# Autodesk Inventor assembly: PnumaticActiveClimb-ver3-1111-2021
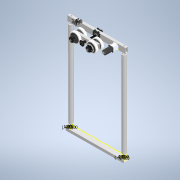
[picture p0: Inventor's stored thumbnail of the model, 180x180]
Saved by Autodesk Inventor 2021 (Build 250183000, 183)
## iProperties
Created: 2021-01-28
Part Number: PnumaticActiveClimb-ver3-1111-2021
Document SubType Name: Assembly
Designer: CMurray
Author: CMurray
## Documents named in this file (19)
- E:\PHRC CADD 2021\PHRC CADD\2020 Infinite Recharge\2021 Infinite Recharge\Chassis\PnumaticActiveClimb-ver3-1111-2021.iam
- E:\PHRC CADD 2021\PHRC CADD\2020 Infinite Recharge\Active Climb\Parts\2x1 16in Aluminum-ver1-1111-2020.ipt
- E:\PHRC CADD 2021\PHRC CADD\Resources\VEXpro Resources\Versa Motion\VersaBlockKit-1111-2016.ipt
- E:\PHRC CADD 2021\PHRC CADD\Resources\VEXpro Resources\Bearings\0.5inHexFlangedBearing(1.125inx0.313in)-1111-2016.ipt
- E:\PHRC CADD 2021\PHRC CADD\Resources\VEXpro Resources\Shafts\0.5inThunderHexShaft(8in(modified))-1111-2016.ipt
- E:\PHRC CADD 2021\PHRC CADD\2020 Infinite Recharge\Active Climb\Parts\AluminumBar-1111-2020.ipt
- E:\PHRC CADD 2021\PHRC CADD\Resources\VEXpro Resources\Spacers\1inAcetalSpacer(0.5inHex)-1111-2016.ipt
- E:\PHRC CADD 2021\PHRC CADD\Resources\VEXpro Resources\Versa Motion\Sprockets\Sprocket15t-ver1-1111-2017.ipt
- E:\PHRC CADD 2021\PHRC CADD\Resources\VEXpro Resources\Versa Motion\Shaft Collars\ClampingShaftCollar0.5inHex-ver1-1111-2017.ipt
- E:\PHRC CADD 2021\PHRC CADD\Resources\VEXpro Resources\Shafts\0.5inThunderHexShaft(8)-1111-2016.ipt
- E:\PHRC CADD 2021\PHRC CADD\Resources\VEXpro Resources\Wheels\4 inch\4inColsonPerformaWheel-1111-2017.ipt
- E:\PHRC CADD 2021\PHRC CADD\Resources\VEXpro Resources\Spacers\.25inchromatesteelwasher-1111-2018.ipt
- E:\PHRC CADD 2021\PHRC CADD\Resources\VEXpro Resources\Versa Motion\Sprockets\1.125HexboreSprocket22t-ver-1111-2018.ipt
- E:\PHRC CADD 2021\PHRC CADD\Resources\VEXpro Resources\Versa Motion\VersaHub(0.5inHex)-1111-2016.ipt
- E:\PHRC CADD 2021\PHRC CADD\Resources\VEXpro Resources\Spacers\0.0625inAcetalSpacer(0.5inHex)-1111-2016.ipt
- E:\PHRC CADD 2021\PHRC CADD\Resources\VEXpro Resources\Spacers\1inAcetalSpacer(0.5inHex)-1111-2016_MIR.ipt
- E:\PHRC CADD 2021\PHRC CADD\Resources\VEXpro Resources\Motors\v2-VersaPlanetary-3in-1stage-with-775pro-20161031.iam
- E:\PHRC CADD 2021\PHRC CADD\2020 Infinite Recharge\Lift\Parts\1.5_Bore_30in_Stroke_ROUND BODY AIR CYLINDER.iam
- E:\PHRC CADD 2021\PHRC CADD\2020 Infinite Recharge\Lift\Assemblies\ClimbBase-1111-2020.iam
## Components (39 placed, 18 different names)
1. 2x1 16in Aluminum-ver1-1111-2020:1 — Rotational:1, Angle:1, Rotational:2, Angle:2, Mate:1, Flush:1, Flush:2, Cylindrical:21, Mate:24, Angle:26, Flush:7, Flush:8, Mate:25
2. VersaBlockKit-1111-2016:1 — Rotational:1, Angle:1, Rotational:3
3. VersaBlockKit-1111-2016:2 — Rotational:2, Angle:2, Rotational:4
4. 0.5inHexFlangedBearing(1.125inx0.313in)-1111-2016:1 — Rotational:3, Cylindrical:1, Angle:6
5. 0.5inHexFlangedBearing(1.125inx0.313in)-1111-2016:2 — Rotational:4, Angle:7
6. 0.5inThunderHexShaft(8in(modified))-1111-2016:1 — Cylindrical:1, Angle:5, Angle:6, Angle:7, Cylindrical:3, Angle:8, Cylindrical:4, Flush:3, Angle:24, Angle:25
7. AluminumBar-1111-2020:1 — Mate:1, Flush:1, Flush:2, Rotational:5, Rotational:6, Flush:3, Rotational:7, Rotational:8, Rotational:9, Rotational:10, Flush:4, Mate:7, Flush:5
8. 0.5inHexFlangedBearing(1.125inx0.313in)-1111-2016:3 — Rotational:5, Cylindrical:2, Mate:2, Angle:3, Angle:4
9. 0.5inHexFlangedBearing(1.125inx0.313in)-1111-2016:4 — Rotational:6, Angle:3, Angle:5
10. 1inAcetalSpacer(0.5inHex)-1111-2016:1 — Cylindrical:2, Mate:2, Angle:4, Mate:3
11. Sprocket15t-ver1-1111-2017:1 — Cylindrical:3, Mate:3, Angle:8, Mate:4
12. ClampingShaftCollar0.5inHex-ver1-1111-2017:1 — Cylindrical:4, Mate:4
13. 0.5inHexFlangedBearing(1.125inx0.313in)-1111-2016:5 — Rotational:7, Cylindrical:5, Angle:9, Mate:17
14. 0.5inHexFlangedBearing(1.125inx0.313in)-1111-2016:6 — Rotational:8, Angle:10, Mate:5
15. 0.5inHexFlangedBearing(1.125inx0.313in)-1111-2016:7 — Rotational:9, Cylindrical:14, Angle:18, Mate:20
16. 0.5inHexFlangedBearing(1.125inx0.313in)-1111-2016:8 — Rotational:10, Angle:19, Mate:18
17. 0.5inThunderHexShaft(8)-1111-2016:1 — Cylindrical:5, Angle:9, Angle:10, Cylindrical:6, Angle:11, Cylindrical:7, Flush:4, Cylindrical:8, Angle:12, Cylindrical:9, Angle:15, Cylindrical:10, Angle:16, Cylindrical:11, Cylindrical:12, Cylindrical:13, Angle:17, Angle:25
18. 4inColsonPerformaWheel-1111-2017:1 — Cylindrical:6, Mate:5, Angle:11, Mate:6
19. .25inchromatesteelwasher-1111-2018:1 — Cylindrical:7, Mate:6
20. 1.125HexboreSprocket22t-ver-1111-2018:1 — Rotational:11, Mate:7, Mate:16
21. VersaHub(0.5inHex)-1111-2016:2 — Rotational:11, Cylindrical:8, Angle:12, Mate:12, Mate:16
22. 0.0625inAcetalSpacer(0.5inHex)-1111-2016:1 — Mate:8, Mate:9, Cylindrical:9, Angle:13, Angle:15, Mate:12
23. 0.0625inAcetalSpacer(0.5inHex)-1111-2016:2 — Mate:8, Mate:9, Mate:10, Mate:11, Angle:13, Angle:14
24. 0.0625inAcetalSpacer(0.5inHex)-1111-2016:3 — Mate:10, Mate:11, Angle:14, Mate:13
25. Sprocket15t-ver1-1111-2017:2 — Cylindrical:10, Angle:16, Mate:13, Mate:14
26. ClampingShaftCollar0.5inHex-ver1-1111-2017:2 — Cylindrical:11, Mate:14, Mate:15
27. .25inchromatesteelwasher-1111-2018:2 — Cylindrical:12, Mate:15
28. 4inColsonPerformaWheel-1111-2017:2 — Cylindrical:13, Mate:17, Angle:17
29. 0.5inThunderHexShaft(8)-1111-2016:2 — Cylindrical:14, Angle:18, Angle:19, Flush:5, Cylindrical:15, Angle:20, Cylindrical:16, Cylindrical:17, Angle:21, Cylindrical:18, Angle:22, Cylindrical:19, Angle:23, Cylindrical:20, Angle:24
30. 4inColsonPerformaWheel-1111-2017:3 — Cylindrical:15, Mate:18, Angle:20, Mate:19
31. .25inchromatesteelwasher-1111-2018:3 — Cylindrical:16, Mate:19
32. 4inColsonPerformaWheel-1111-2017:4 — Cylindrical:17, Mate:20, Angle:21, Mate:21
33. 1inAcetalSpacer(0.5inHex)-1111-2016_MIR:1 — Cylindrical:18, Mate:21, Angle:22, Mate:22
34. Sprocket15t-ver1-1111-2017:3 — Cylindrical:19, Mate:22, Angle:23, Mate:23
35. .25inchromatesteelwasher-1111-2018:4 — Cylindrical:20, Mate:23
36. v2-VersaPlanetary-3in-1stage-with-775pro-20161031:1 [sub-assembly] — Cylindrical:21, Mate:24, Angle:26
37. 1.5_Bore_30in_Stroke_ROUND BODY AIR CYLINDER:3 [sub-assembly] — Flush:6
38. 1.5_Bore_30in_Stroke_ROUND BODY AIR CYLINDER:4 [sub-assembly] — Rotational:12, Flush:6
39. ClimbBase-1111-2020:2 [sub-assembly] — Rotational:12, Flush:7, Flush:8, Mate:25
## Relationships (93: Angle 26, Mate 25, CylindricalJoint 21, RevoluteJoint 12, Flush 8, Insert 1)
- Rotational:1 [RevoluteJoint]: 2x1 16in Aluminum-ver1-1111-2020:1 ↔ VersaBlockKit-1111-2016:1
- Angle:1 (0 deg): 2x1 16in Aluminum-ver1-1111-2020:1 ↔ VersaBlockKit-1111-2016:1
- Rotational:2 [RevoluteJoint]: 2x1 16in Aluminum-ver1-1111-2020:1 ↔ VersaBlockKit-1111-2016:2
- Angle:2 (0 deg): 2x1 16in Aluminum-ver1-1111-2020:1 ↔ VersaBlockKit-1111-2016:2
- Rotational:3 [RevoluteJoint]: VersaBlockKit-1111-2016:1 ↔ 0.5inHexFlangedBearing(1.125inx0.313in)-1111-2016:1
- Rotational:4 [RevoluteJoint]: VersaBlockKit-1111-2016:2 ↔ 0.5inHexFlangedBearing(1.125inx0.313in)-1111-2016:2
- Cylindrical:1: 0.5inHexFlangedBearing(1.125inx0.313in)-1111-2016:1 ↔ 0.5inThunderHexShaft(8in(modified))-1111-2016:1
- Mate:1 (85.725 mm): 2x1 16in Aluminum-ver1-1111-2020:1 ↔ AluminumBar-1111-2020:1
- Flush:1: 2x1 16in Aluminum-ver1-1111-2020:1 ↔ AluminumBar-1111-2020:1
- Flush:2 (174.625 mm): 2x1 16in Aluminum-ver1-1111-2020:1 ↔ AluminumBar-1111-2020:1
- Rotational:5 [RevoluteJoint]: AluminumBar-1111-2020:1 ↔ 0.5inHexFlangedBearing(1.125inx0.313in)-1111-2016:3
- Rotational:6 [RevoluteJoint]: AluminumBar-1111-2020:1 ↔ 0.5inHexFlangedBearing(1.125inx0.313in)-1111-2016:4
- Cylindrical:2: 0.5inHexFlangedBearing(1.125inx0.313in)-1111-2016:3 ↔ 1inAcetalSpacer(0.5inHex)-1111-2016:1
- Mate:2: 0.5inHexFlangedBearing(1.125inx0.313in)-1111-2016:3 ↔ 1inAcetalSpacer(0.5inHex)-1111-2016:1
- Angle:3 (0 deg): 0.5inHexFlangedBearing(1.125inx0.313in)-1111-2016:3 ↔ 0.5inHexFlangedBearing(1.125inx0.313in)-1111-2016:4
- Angle:4 (0 deg): 0.5inHexFlangedBearing(1.125inx0.313in)-1111-2016:3 ↔ 1inAcetalSpacer(0.5inHex)-1111-2016:1
- Angle:5 (90 deg): 0.5inThunderHexShaft(8in(modified))-1111-2016:1 ↔ 0.5inHexFlangedBearing(1.125inx0.313in)-1111-2016:4
- Angle:6 (90 deg): 0.5inHexFlangedBearing(1.125inx0.313in)-1111-2016:1 ↔ 0.5inThunderHexShaft(8in(modified))-1111-2016:1
- Angle:7 (90 deg): 0.5inHexFlangedBearing(1.125inx0.313in)-1111-2016:2 ↔ 0.5inThunderHexShaft(8in(modified))-1111-2016:1
- Cylindrical:3: 0.5inThunderHexShaft(8in(modified))-1111-2016:1 ↔ Sprocket15t-ver1-1111-2017:1
- Mate:3: 1inAcetalSpacer(0.5inHex)-1111-2016:1 ↔ Sprocket15t-ver1-1111-2017:1
- Angle:8 (90 deg): 0.5inThunderHexShaft(8in(modified))-1111-2016:1 ↔ Sprocket15t-ver1-1111-2017:1
- Cylindrical:4: 0.5inThunderHexShaft(8in(modified))-1111-2016:1 ↔ ClampingShaftCollar0.5inHex-ver1-1111-2017:1
- Mate:4: Sprocket15t-ver1-1111-2017:1 ↔ ClampingShaftCollar0.5inHex-ver1-1111-2017:1
- Flush:3 (50.8 mm): 0.5inThunderHexShaft(8in(modified))-1111-2016:1 ↔ AluminumBar-1111-2020:1
- Rotational:7 [RevoluteJoint]: AluminumBar-1111-2020:1 ↔ 0.5inHexFlangedBearing(1.125inx0.313in)-1111-2016:5
- Rotational:8 [RevoluteJoint]: AluminumBar-1111-2020:1 ↔ 0.5inHexFlangedBearing(1.125inx0.313in)-1111-2016:6
- Rotational:9 [RevoluteJoint]: AluminumBar-1111-2020:1 ↔ 0.5inHexFlangedBearing(1.125inx0.313in)-1111-2016:7
- Rotational:10 [RevoluteJoint]: AluminumBar-1111-2020:1 ↔ 0.5inHexFlangedBearing(1.125inx0.313in)-1111-2016:8
- Cylindrical:5: 0.5inHexFlangedBearing(1.125inx0.313in)-1111-2016:5 ↔ 0.5inThunderHexShaft(8)-1111-2016:1
- Angle:9 (90 deg): 0.5inHexFlangedBearing(1.125inx0.313in)-1111-2016:5 ↔ 0.5inThunderHexShaft(8)-1111-2016:1
- Angle:10 (90 deg): 0.5inHexFlangedBearing(1.125inx0.313in)-1111-2016:6 ↔ 0.5inThunderHexShaft(8)-1111-2016:1
- Cylindrical:6: 0.5inThunderHexShaft(8)-1111-2016:1 ↔ 4inColsonPerformaWheel-1111-2017:1
- Mate:5: 0.5inHexFlangedBearing(1.125inx0.313in)-1111-2016:6 ↔ 4inColsonPerformaWheel-1111-2017:1
- Angle:11 (90 deg): 0.5inThunderHexShaft(8)-1111-2016:1 ↔ 4inColsonPerformaWheel-1111-2017:1
- Cylindrical:7: 0.5inThunderHexShaft(8)-1111-2016:1 ↔ .25inchromatesteelwasher-1111-2018:1
- Mate:6: 4inColsonPerformaWheel-1111-2017:1 ↔ .25inchromatesteelwasher-1111-2018:1
- Flush:4 (38.1 mm): AluminumBar-1111-2020:1 ↔ 0.5inThunderHexShaft(8)-1111-2016:1
- Rotational:11 [RevoluteJoint]: 1.125HexboreSprocket22t-ver-1111-2018:1 ↔ VersaHub(0.5inHex)-1111-2016:2
- Cylindrical:8: 0.5inThunderHexShaft(8)-1111-2016:1 ↔ VersaHub(0.5inHex)-1111-2016:2
- Mate:7 (34.925 mm): AluminumBar-1111-2020:1 ↔ 1.125HexboreSprocket22t-ver-1111-2018:1
- Mate:8: 0.0625inAcetalSpacer(0.5inHex)-1111-2016:1 ↔ 0.0625inAcetalSpacer(0.5inHex)-1111-2016:2
- Mate:9: 0.0625inAcetalSpacer(0.5inHex)-1111-2016:1 ↔ 0.0625inAcetalSpacer(0.5inHex)-1111-2016:2
- Mate:10: 0.0625inAcetalSpacer(0.5inHex)-1111-2016:2 ↔ 0.0625inAcetalSpacer(0.5inHex)-1111-2016:3
- Mate:11: 0.0625inAcetalSpacer(0.5inHex)-1111-2016:2 ↔ 0.0625inAcetalSpacer(0.5inHex)-1111-2016:3
- Angle:12 (90 deg): 0.5inThunderHexShaft(8)-1111-2016:1 ↔ VersaHub(0.5inHex)-1111-2016:2
- Cylindrical:9: 0.5inThunderHexShaft(8)-1111-2016:1 ↔ 0.0625inAcetalSpacer(0.5inHex)-1111-2016:1
- Angle:13 (0 deg): 0.0625inAcetalSpacer(0.5inHex)-1111-2016:1 ↔ 0.0625inAcetalSpacer(0.5inHex)-1111-2016:2
- Angle:14 (90 deg): 0.0625inAcetalSpacer(0.5inHex)-1111-2016:2 ↔ 0.0625inAcetalSpacer(0.5inHex)-1111-2016:3
- Angle:15 (90 deg): 0.5inThunderHexShaft(8)-1111-2016:1 ↔ 0.0625inAcetalSpacer(0.5inHex)-1111-2016:1
- Mate:12: VersaHub(0.5inHex)-1111-2016:2 ↔ 0.0625inAcetalSpacer(0.5inHex)-1111-2016:1
- Cylindrical:10: 0.5inThunderHexShaft(8)-1111-2016:1 ↔ Sprocket15t-ver1-1111-2017:2
- Angle:16 (90 deg): 0.5inThunderHexShaft(8)-1111-2016:1 ↔ Sprocket15t-ver1-1111-2017:2
- Mate:13: 0.0625inAcetalSpacer(0.5inHex)-1111-2016:3 ↔ Sprocket15t-ver1-1111-2017:2
- Cylindrical:11: 0.5inThunderHexShaft(8)-1111-2016:1 ↔ ClampingShaftCollar0.5inHex-ver1-1111-2017:2
- Mate:14: Sprocket15t-ver1-1111-2017:2 ↔ ClampingShaftCollar0.5inHex-ver1-1111-2017:2
- Cylindrical:12: 0.5inThunderHexShaft(8)-1111-2016:1 ↔ .25inchromatesteelwasher-1111-2018:2
- Mate:15: ClampingShaftCollar0.5inHex-ver1-1111-2017:2 ↔ .25inchromatesteelwasher-1111-2018:2
- Mate:16: 1.125HexboreSprocket22t-ver-1111-2018:1 ↔ VersaHub(0.5inHex)-1111-2016:2
- Cylindrical:13: 0.5inThunderHexShaft(8)-1111-2016:1 ↔ 4inColsonPerformaWheel-1111-2017:2
- Mate:17: 0.5inHexFlangedBearing(1.125inx0.313in)-1111-2016:5 ↔ 4inColsonPerformaWheel-1111-2017:2
- Angle:17 (90 deg): 0.5inThunderHexShaft(8)-1111-2016:1 ↔ 4inColsonPerformaWheel-1111-2017:2
- Cylindrical:14: 0.5inHexFlangedBearing(1.125inx0.313in)-1111-2016:7 ↔ 0.5inThunderHexShaft(8)-1111-2016:2
- Angle:18 (90 deg): 0.5inHexFlangedBearing(1.125inx0.313in)-1111-2016:7 ↔ 0.5inThunderHexShaft(8)-1111-2016:2
- Angle:19 (90 deg): 0.5inHexFlangedBearing(1.125inx0.313in)-1111-2016:8 ↔ 0.5inThunderHexShaft(8)-1111-2016:2
- Flush:5 (-38.1 mm): AluminumBar-1111-2020:1 ↔ 0.5inThunderHexShaft(8)-1111-2016:2
- Cylindrical:15: 0.5inThunderHexShaft(8)-1111-2016:2 ↔ 4inColsonPerformaWheel-1111-2017:3
- Mate:18: 0.5inHexFlangedBearing(1.125inx0.313in)-1111-2016:8 ↔ 4inColsonPerformaWheel-1111-2017:3
- Angle:20 (0 deg): 0.5inThunderHexShaft(8)-1111-2016:2 ↔ 4inColsonPerformaWheel-1111-2017:3
- Cylindrical:16: 0.5inThunderHexShaft(8)-1111-2016:2 ↔ .25inchromatesteelwasher-1111-2018:3
- Mate:19: 4inColsonPerformaWheel-1111-2017:3 ↔ .25inchromatesteelwasher-1111-2018:3
- Cylindrical:17: 0.5inThunderHexShaft(8)-1111-2016:2 ↔ 4inColsonPerformaWheel-1111-2017:4
- Mate:20: 0.5inHexFlangedBearing(1.125inx0.313in)-1111-2016:7 ↔ 4inColsonPerformaWheel-1111-2017:4
- Angle:21 (90 deg): 0.5inThunderHexShaft(8)-1111-2016:2 ↔ 4inColsonPerformaWheel-1111-2017:4
- Cylindrical:18: 0.5inThunderHexShaft(8)-1111-2016:2 ↔ 1inAcetalSpacer(0.5inHex)-1111-2016_MIR:1
- Mate:21: 4inColsonPerformaWheel-1111-2017:4 ↔ 1inAcetalSpacer(0.5inHex)-1111-2016_MIR:1
- Angle:22 (90 deg): 0.5inThunderHexShaft(8)-1111-2016:2 ↔ 1inAcetalSpacer(0.5inHex)-1111-2016_MIR:1
- Cylindrical:19: 0.5inThunderHexShaft(8)-1111-2016:2 ↔ Sprocket15t-ver1-1111-2017:3
- Mate:22: 1inAcetalSpacer(0.5inHex)-1111-2016_MIR:1 ↔ Sprocket15t-ver1-1111-2017:3
- Angle:23 (90 deg): 0.5inThunderHexShaft(8)-1111-2016:2 ↔ Sprocket15t-ver1-1111-2017:3
- Cylindrical:20: 0.5inThunderHexShaft(8)-1111-2016:2 ↔ .25inchromatesteelwasher-1111-2018:4
- Mate:23: Sprocket15t-ver1-1111-2017:3 ↔ .25inchromatesteelwasher-1111-2018:4
- Angle:24 (0 deg): 0.5inThunderHexShaft(8in(modified))-1111-2016:1 ↔ 0.5inThunderHexShaft(8)-1111-2016:2
- Angle:25 (0 deg): 0.5inThunderHexShaft(8in(modified))-1111-2016:1 ↔ 0.5inThunderHexShaft(8)-1111-2016:1
- Cylindrical:21: 2x1 16in Aluminum-ver1-1111-2020:1 ↔ v2-VersaPlanetary-3in-1stage-with-775pro-20161031:1
- Mate:24: 2x1 16in Aluminum-ver1-1111-2020:1 ↔ v2-VersaPlanetary-3in-1stage-with-775pro-20161031:1
- Angle:26 (0 deg): 2x1 16in Aluminum-ver1-1111-2020:1 ↔ v2-VersaPlanetary-3in-1stage-with-775pro-20161031:1
- [Insert]: 1.5_Bore_30in_Stroke_ROUND BODY AIR CYLINDER:3 ↔ ClimbBase-1111-2020:2
- Rotational:12 [RevoluteJoint]: 1.5_Bore_30in_Stroke_ROUND BODY AIR CYLINDER:4 ↔ ClimbBase-1111-2020:2
- Flush:6: 1.5_Bore_30in_Stroke_ROUND BODY AIR CYLINDER:3 ↔ 1.5_Bore_30in_Stroke_ROUND BODY AIR CYLINDER:4
- Flush:7: 2x1 16in Aluminum-ver1-1111-2020:1 ↔ ClimbBase-1111-2020:2
- Flush:8: 2x1 16in Aluminum-ver1-1111-2020:1 ↔ ClimbBase-1111-2020:2
- Mate:25 (889.635 mm): 2x1 16in Aluminum-ver1-1111-2020:1 ↔ ClimbBase-1111-2020:2
